# Autodesk Inventor assembly: Ring
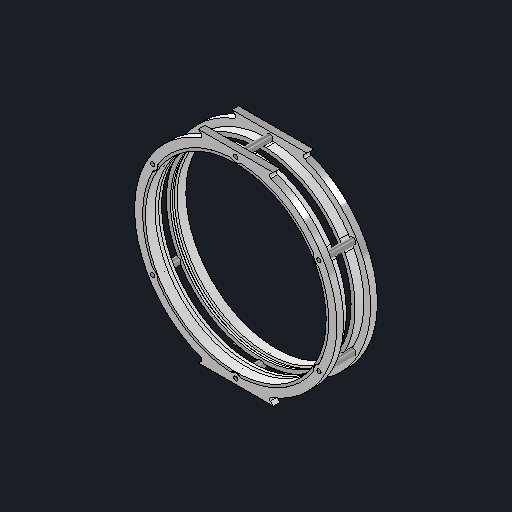
[picture p0: Inventor's stored thumbnail of the model, 512x512]
Saved by Autodesk Inventor 2023.2 (Build 272271030, 271C)
## iProperties
Created: 2024-02-21
Part Number: Ring
Document SubType Name: Assembly
Designer: robpl
Mass: 88.972 g
Surface Area: 226.523 cm^2
Volume: 27.4949 cm^3
Density: 3.23594 g/cm^3
Author: robpl
## Documents named in this file (5)
- C:\Users\robpl\OneDrive\Documents\Arduino\Onslaught\CAD\Frame Test\Ring.iam
- C:\Users\robpl\OneDrive\Documents\Arduino\Onslaught\CAD\Frame Test\Weapon Disk.ipt
- C:\Users\robpl\OneDrive\Documents\Arduino\Onslaught\CAD\Frame Test\Pin.ipt
- C:\Users\robpl\OneDrive\Documents\Arduino\Onslaught\CAD\Frame Test\Ring Bearing Track.ipt
- C:\Users\robpl\OneDrive\Documents\Arduino\Onslaught\CAD\Frame Test\Ring Driving Track.ipt
## Components (10 placed, 4 different names)
1. Weapon Disk:1 — Mate:1, Mate:3, Flush:1, Mate:5, Mate:6
2. Weapon Disk:2 — Mate:1, Mate:3, Mate:4, Mate:8, Mate:9
3. Ring Bearing Track:1 — Mate:5, Mate:6, Mate:7
4. Ring Driving Track:1 — Mate:8, Mate:9, Mate:10
5. Pin:1 — Mate:4, Flush:1
6. Pin:2 — Mate:7
7. Pin:3 — Mate:10
8. Pin:4
9. Pin:5
10. Pin:6
## Component patterns: (6 elements, first: Pin:1)
## Relationships (10: Mate 9, Flush 1)
- Mate:1: Weapon Disk:1 ↔ Weapon Disk:2
- Mate:3 (20 mm): Weapon Disk:1 ↔ Weapon Disk:2
- Mate:4: Weapon Disk:2 ↔ Pin:1
- Flush:1: Weapon Disk:1 ↔ Pin:1
- Mate:5: Weapon Disk:1 ↔ Ring Bearing Track:1
- Mate:6: Weapon Disk:1 ↔ Ring Bearing Track:1
- Mate:7: Ring Bearing Track:1 ↔ Pin:2
- Mate:8: Weapon Disk:2 ↔ Ring Driving Track:1
- Mate:9: Weapon Disk:2 ↔ Ring Driving Track:1
- Mate:10: Ring Driving Track:1 ↔ Pin:3
